# Autodesk Inventor assembly: HaptHexa_leg_r2
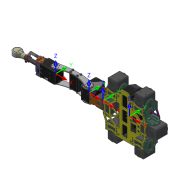
[picture p0: Inventor's stored thumbnail of the model, 180x180]
Saved by Autodesk Inventor 2019.4 (Build 234330000, 330)
## iProperties
Created: 2018-12-18
Part Number: HaptHexa_leg_r2
Material: 一般
Document SubType Name: Assembly
Designer: y6tada
Mass: 2067.58 g
Surface Area: 7353.68 cm^2
Volume: 1514.35 cm^3
Density: 1.36532 g/cm^3
Author: y6tada
## Documents named in this file (7)
- C:\Workspace\HaptHexa\Hardware\Inventor\HaptHexa_leg_r2.iam
- C:\Workspace\HaptHexa\Hardware\Inventor\Thorax\_Thorax.iam
- C:\Workspace\HaptHexa\Hardware\Inventor\Coxa\_Coxa.iam
- C:\Workspace\HaptHexa\Hardware\Inventor\Femur\_Femur.iam
- C:\Workspace\HaptHexa\Hardware\Inventor\Tibia\_Tibia.iam
- C:\Workspace\HaptHexa\Hardware\Inventor\Computer\_Computer.iam
- C:\Workspace\HaptHexa\Hardware\Inventor\Computer\Intel Realsense D435\D435_ipt.ipt
## Components (6 placed, 6 different names)
1. _Thorax:1 [sub-assembly] — メイト:11, メイト:12, 角度:2
2. _Computer:1 [sub-assembly] — フラッシュ:1, フラッシュ:2, 角度:4
3. D435_ipt:1 — フラッシュ:2, 角度:4
4. _Coxa:2 [sub-assembly] — メイト:11, メイト:12, 角度:2, メイト:48, メイト:49, 角度:5
5. _Femur:2 [sub-assembly] — メイト:48, メイト:49, メイト:50, メイト:51, 角度:5, 角度:6
6. _Tibia:2 [sub-assembly] — メイト:50, メイト:51, 角度:6
## Relationships (13: Mate 6, Angle 4, Flush 3)
- 角度:2 [Angle] (180 deg): _Thorax:1 ↔ _Coxa:2
- メイト:11 [Mate]: _Thorax:1 ↔ _Coxa:2
- メイト:12 [Mate]: _Thorax:1 ↔ _Coxa:2
- フラッシュ:1 [Flush]: _Computer:1
- フラッシュ:2 [Flush]: _Computer:1 ↔ D435_ipt:1
- 角度:4 [Angle] (-35 deg): _Computer:1 ↔ D435_ipt:1
- メイト:48 [Mate]: _Coxa:2 ↔ _Femur:2
- メイト:49 [Mate]: _Coxa:2 ↔ _Femur:2
- メイト:50 [Mate]: _Femur:2 ↔ _Tibia:2
- メイト:51 [Mate]: _Femur:2 ↔ _Tibia:2
- フラッシュ:3 [Flush] (-80 mm)
- 角度:5 [Angle] (0 deg): _Coxa:2 ↔ _Femur:2
- 角度:6 [Angle] (0 deg): _Femur:2 ↔ _Tibia:2
## Named parameters: femur_angle = 0 deg, tibia_angle = 0 deg
